# Autodesk Inventor assembly: arm
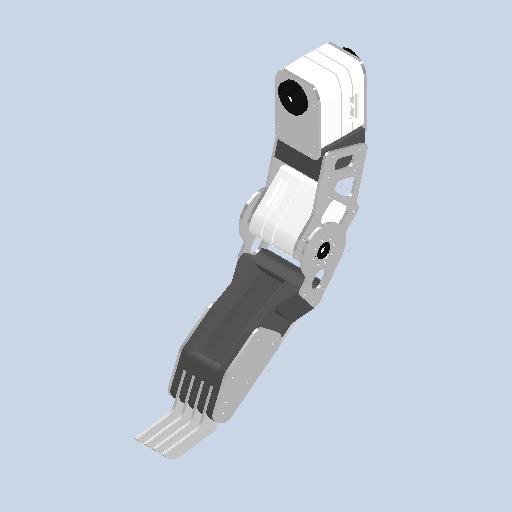
[picture p0: Inventor's stored thumbnail of the model, 512x512]
Saved by Autodesk Inventor 2024.1 (Build 281209000, 209)
## iProperties
Created: 2024-02-14
Part Number: arm
Document SubType Name: Assembly
Designer: hibik
Author: hibik
## Documents named in this file (7)
- C:\Users\hibik\Desktop\ロボメカ\HR\2024.02.11 Rl\02.11 ProtType\arm.iam
- C:\Users\hibik\Desktop\ロボメカ\HR\2024.02.11 Rl\KRS3300モータ.ipt
- C:\Users\hibik\Desktop\ロボメカ\HR\2024.02.11 Rl\02.11 ProtType\arm.ipt
- C:\Users\hibik\Desktop\ロボメカ\HR\2024.02.11 Rl\02.11 ProtType\arm_middle.ipt
- C:\Users\hibik\Desktop\ロボメカ\HR\2024.02.11 Rl\KRS3300サーボホーン.ipt
- C:\Users\hibik\Desktop\ロボメカ\HR\2024.02.11 Rl\02.11 ProtType\elbow.ipt
- C:\Users\hibik\Desktop\ロボメカ\HR\2024.02.11 Rl\02.11 ProtType\hand.iam
## Components (12 placed, 6 different names)
1. KRS3300モータ:1 — 挿入:1, 挿入:2, 角度:1, 角度:2, 挿入:5, 挿入:6
2. arm:1 — 挿入:1, 角度:1, 挿入:12, 挿入:13
3. arm:2 — 挿入:2, 角度:2
4. arm_middle:1 — 挿入:12, 挿入:13, 挿入:16, 挿入:17, 挿入:18, 挿入:19
5. KRS3300サーボホーン:1 — 挿入:5
6. KRS3300サーボホーン:2 — 挿入:6
7. KRS3300モータ:2 — 挿入:14, 挿入:15, 挿入:20, 角度:3
8. KRS3300サーボホーン:3 — 挿入:15, 挿入:21
9. KRS3300サーボホーン:4 — 挿入:14
10. elbow:1 — 挿入:16, 挿入:17, 挿入:20, 角度:3
11. elbow:2 — 挿入:18, 挿入:19
12. hand:1 [sub-assembly] — 挿入:21
## Relationships (17: Insert 14, Angle 3)
- 挿入:1 [Insert]: KRS3300モータ:1 ↔ arm:1
- 挿入:2 [Insert]: KRS3300モータ:1 ↔ arm:2
- 角度:1 [Angle] (0 deg): KRS3300モータ:1 ↔ arm:1
- 角度:2 [Angle] (0 deg): KRS3300モータ:1 ↔ arm:2
- 挿入:5 [Insert] (0.3 mm): KRS3300モータ:1 ↔ KRS3300サーボホーン:1
- 挿入:6 [Insert] (0.3 mm): KRS3300モータ:1 ↔ KRS3300サーボホーン:2
- 挿入:12 [Insert]: arm:1 ↔ arm_middle:1
- 挿入:13 [Insert]: arm:1 ↔ arm_middle:1
- 挿入:14 [Insert] (0.3 mm): KRS3300モータ:2 ↔ KRS3300サーボホーン:4
- 挿入:15 [Insert] (0.3 mm): KRS3300モータ:2 ↔ KRS3300サーボホーン:3
- 挿入:16 [Insert]: arm_middle:1 ↔ elbow:1
- 挿入:17 [Insert]: arm_middle:1 ↔ elbow:1
- 挿入:18 [Insert]: arm_middle:1 ↔ elbow:2
- 挿入:19 [Insert]: arm_middle:1 ↔ elbow:2
- 挿入:20 [Insert]: KRS3300モータ:2 ↔ elbow:1
- 角度:3 [Angle] (0 deg): KRS3300モータ:2 ↔ elbow:1
- 挿入:21 [Insert]: KRS3300サーボホーン:3 ↔ hand:1
